# Autodesk Inventor assembly: AM14U2_Square
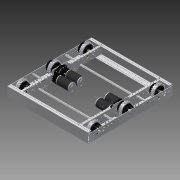
[picture p0: Inventor's stored thumbnail of the model, 180x180]
Saved by Autodesk Inventor 2015 SP1 (Build 190203100, 203)
## iProperties
Category: Drive Base
Company: Autodesk Inc.
Created: 2014-12-16
Part Number: AM14U2_Square
Document SubType Name: Assembly
Designer: Autodesk Inc.
Catalog Web Link: andymark.com
Vendor: Andy Mark Inc.
Author: Autodesk Inc.
## Documents named in this file (2)
- C:\FRC_KOP_2015_Test\Drive Base\DB_DriveBaseSquare_AM14U2.iam
- C:\FRC_KOP_2015_Test\Drive Base\Parts\AM14U2 Half Square.iam
## Components (2 placed, 2 different names)
1. AM14U2 Half Square_1 [sub-assembly] — Insert:1
2. AM14U2 Half Square_2 [sub-assembly] — Insert:1
## Relationships (1: Insert 1)
- Insert:1: AM14U2 Half Square_1 ↔ AM14U2 Half Square_2
